# Autodesk Inventor assembly: StopMechanismAssembly
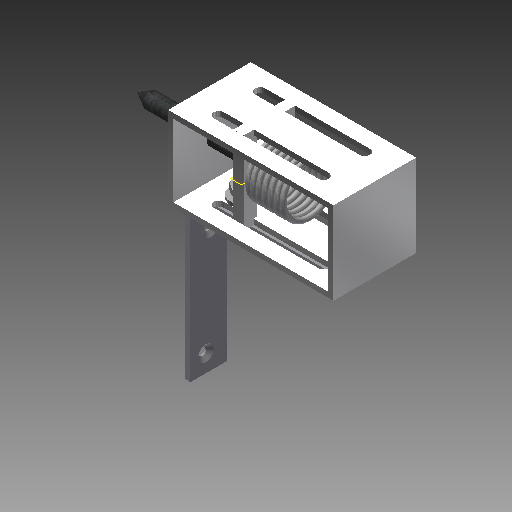
[picture p0: Inventor's stored thumbnail of the model, 512x512]
Saved by Autodesk Inventor 2017.2 (Build 212233000, 233)
## iProperties
Created: 2016-02-17
Part Number: StopMechanismAssembly
Document SubType Name: Assembly
Designer: steele
Mass: 221.776 g
Surface Area: 431.604 cm^2
Volume: 61.0209 cm^3
Density: 3.63442 g/cm^3
Author: steele
## Documents named in this file (9)
- D:\snobotics\CAD-Development\robSteele\SnoBotics2016\2016-02-17-StopMechanism\StopMechanismAssembly.iam
- D:\snobotics\CAD-Development\robSteele\SnoBotics2016\2016-02-17-StopMechanism\StopMechanismHousing.ipt
- D:\snobotics\CAD-Development\robSteele\SnoBotics2016\2016-02-17-StopMechanism\outerTubeStopPost.ipt
- D:\snobotics\CAD-Development\robSteele\SnoBotics2016\2016-02-17-StopMechanism\StopMechanismPushPlate.ipt
- D:\snobotics\CAD-Development\robSteele\SnoBotics2016\2016-02-17-StopMechanism\StopMechanismAssembly\Design Accelerator\Compress Spring1.iam
- D:\snobotics\CAD-Development\robSteele\SnoBotics2016\2016-02-17-StopMechanism\StopMechanismAssembly\Design Accelerator\Bolted Connection1.iam
- D:\snobotics\CAD-MfgResources\McMaster-Carr\Bracket\4 Inch\1556A170.ipt
- D:\snobotics\CAD-Development\robSteele\SnoBotics2016\2016-02-17-StopMechanism\StopMechanismAssembly\Design Accelerator\Bolted Connection3.iam
- D:\snobotics\CAD-Development\robSteele\SnoBotics2016\2016-02-17-StopMechanism\StopMechanismAssembly\Design Accelerator\Bolted Connection4.iam
## Components (8 placed, 6 different names)
1. StopMechanismHousing:1 — Insert:1, Mate:4, Flush:2, Flush:3
2. outerTubeStopPost:1 — Insert:1, Insert:2, Mate:10
3. StopMechanismPushPlate:1 — Mate:1, Flush:1, Insert:2, Mate:9
4. Compress Spring:1 [sub-assembly] — Mate:1, Flush:1
5. Bolted Connection:1 [sub-assembly] — Mate:9, Mate:10
6. 1556A170:1 — Mate:4, Flush:2, Flush:3, Mate:5, Mate:6, Mate:7, Mate:8
7. Bolted Connection:2 [sub-assembly] — Mate:5, Mate:6
8. Bolted Connection:3 [sub-assembly] — Mate:7, Mate:8
## Relationships (13: Mate 8, Flush 3, Insert 2)
- Mate:1: StopMechanismPushPlate:1 ↔ Compress Spring:1
- Flush:1: StopMechanismPushPlate:1 ↔ Compress Spring:1
- Insert:1 (-30.48 mm): StopMechanismHousing:1 ↔ outerTubeStopPost:1
- Insert:2: outerTubeStopPost:1 ↔ StopMechanismPushPlate:1
- Mate:4: StopMechanismHousing:1 ↔ 1556A170:1
- Flush:2 (-3.683 mm): StopMechanismHousing:1 ↔ 1556A170:1
- Flush:3 (-14.2875 mm): StopMechanismHousing:1 ↔ 1556A170:1
- Mate:5: 1556A170:1 ↔ Bolted Connection:2
- Mate:6: 1556A170:1 ↔ Bolted Connection:2
- Mate:7: 1556A170:1 ↔ Bolted Connection:3
- Mate:8: 1556A170:1 ↔ Bolted Connection:3
- Mate:9: StopMechanismPushPlate:1 ↔ Bolted Connection:1
- Mate:10: outerTubeStopPost:1 ↔ Bolted Connection:1
